# Autodesk Inventor assembly: DustDetector
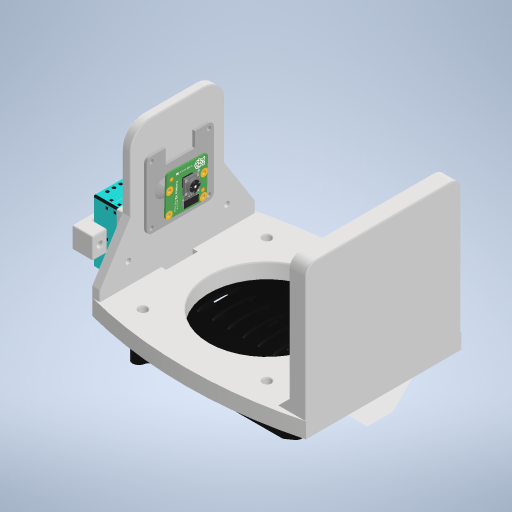
[picture p0: Inventor's stored thumbnail of the model, 512x512]
Saved by Autodesk Inventor 2024.2 (Build 282272000, 272)
## iProperties
Created: 2023-08-29
Part Number: DustDetector
Document SubType Name: Assembly
Designer: N. Spada
Author: N. Spada
## Documents named in this file (9)
- G:\My Drive\Design\NSpadaCAD\DustDetector\DustDetector.iam
- G:\My Drive\Design\NSpadaCAD\DustDetector\pi4_bottom.ipt
- G:\My Drive\Design\NSpadaCAD\DustDetector\cameraMountv4_NS.ipt
- G:\My Drive\Design\NSpadaCAD\DustDetector\pi4_cover_40mm.ipt
- G:\My Drive\Design\NSpadaCAD\DustDetector\LightPad.ipt
- G:\My Drive\Design\NSpadaCAD\DustDetector\Cam V2.1 v1\Cam V2.1 v1.ipt
- G:\My Drive\Design\NSpadaCAD\DustDetector\PMS5003\PMS5003.ipt
- G:\My Drive\Design\NSpadaCAD\DustDetector\Stand.ipt
- G:\My Drive\Design\NSpadaCAD\DustDetector\PMSretainer.ipt
## Components (8 placed, 8 different names)
1. pi4_bottom:1 — Flush:1, Flush:2, Mate:1, Mate:12, Mate:13
2. cameraMountv4_NS:1 — Mate:2, Mate:3, Mate:9, Mate:10, Mate:11
3. pi4_cover_40mm:1 — Flush:1, Flush:2, Mate:1
4. LightPad:1 — Mate:4, Mate:5, Mate:6
5. Cam V2.1 v1:1 — Mate:2, Mate:3
6. PMS5003:1 — Mate:14, Flush:5, Mate:15, Mate:16
7. Stand:1 — Mate:4, Mate:5, Mate:6, Flush:3, Flush:4, Mate:7, Mate:9, Mate:10, Mate:11, Mate:12, Mate:13, Mate:14, Flush:5, Mate:15, Mate:17, Mate:18
8. PMSretainer:1 — Mate:16, Mate:17, Mate:18
## Relationships (22: Mate 17, Flush 5)
- Flush:1: pi4_bottom:1 ↔ pi4_cover_40mm:1
- Flush:2: pi4_bottom:1 ↔ pi4_cover_40mm:1
- Mate:1: pi4_bottom:1 ↔ pi4_cover_40mm:1
- Mate:2: cameraMountv4_NS:1 ↔ Cam V2.1 v1:1
- Mate:3: cameraMountv4_NS:1 ↔ Cam V2.1 v1:1
- Mate:4: LightPad:1 ↔ Stand:1
- Mate:5: LightPad:1 ↔ Stand:1
- Mate:6: LightPad:1 ↔ Stand:1
- Flush:3: Stand:1
- Flush:4: Stand:1
- Mate:7: Stand:1
- Mate:9: cameraMountv4_NS:1 ↔ Stand:1
- Mate:10: cameraMountv4_NS:1 ↔ Stand:1
- Mate:11: cameraMountv4_NS:1 ↔ Stand:1
- Mate:12: pi4_bottom:1 ↔ Stand:1
- Mate:13: pi4_bottom:1 ↔ Stand:1
- Mate:14: PMS5003:1 ↔ Stand:1
- Flush:5: PMS5003:1 ↔ Stand:1
- Mate:15: PMS5003:1 ↔ Stand:1
- Mate:16: PMS5003:1 ↔ PMSretainer:1
- Mate:17: Stand:1 ↔ PMSretainer:1
- Mate:18: Stand:1 ↔ PMSretainer:1
